# Autodesk Inventor assembly: Assembly_Cube_Lens_holder_v3
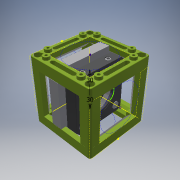
[picture p0: Inventor's stored thumbnail of the model, 180x180]
Saved by Autodesk Inventor 2019 (Build 230136000, 136)
## iProperties
Created: 2020-11-11
Part Number: Assembly_Cube_Lens_holder_v3
Document SubType Name: Assembly
Designer: marsikovabarbora
Author: marsikovabarbora
## Documents named in this file (4)
- C:\Users\UC2\Dropbox\UC2\02_CAD\INVENTOR\uc2_v3\Assembly_Cube_Thorlabs_Cage_v3.iam
- C:\Users\UC2\Dropbox\UC2\02_CAD\INVENTOR\uc2_v3\Assembly_Cube_empty_IM_v3.iam
- C:\Users\UC2\Dropbox\UC2\02_CAD\INVENTOR\uc2_v3\00_Thorlabs_Cage_CP33_M.ipt
- C:\Users\UC2\Dropbox\UC2\02_CAD\INVENTOR\uc2_v3\Imported Components\20_Insert_Thorlabs_holder_v3\20_Insert_Thorlabs_holder_v3.ipt
## Components (3 placed, 3 different names)
1. Assembly_Cube_empty_IM_v3:1 [sub-assembly] — Mate:1, Mate:2, Mate:3, Passend:5, Passend:6, Winkel:2
2. 00_Thorlabs_Cage_CP33_M:1 — Passend:4, Winkel:1, Fluchtend:1
3. 20_Insert_Thorlabs_holder_v3:1 — Passend:4, Winkel:1, Fluchtend:1, Passend:5, Passend:6, Winkel:2
## Relationships (9: Mate 6, Angle 2, Flush 1)
- Mate:1: Assembly_Cube_empty_IM_v3:1
- Mate:2: Assembly_Cube_empty_IM_v3:1
- Mate:3: Assembly_Cube_empty_IM_v3:1
- Passend:4 [Mate]: 00_Thorlabs_Cage_CP33_M:1 ↔ 20_Insert_Thorlabs_holder_v3:1
- Winkel:1 [Angle] (0 deg): 00_Thorlabs_Cage_CP33_M:1 ↔ 20_Insert_Thorlabs_holder_v3:1
- Fluchtend:1 [Flush]: 00_Thorlabs_Cage_CP33_M:1 ↔ 20_Insert_Thorlabs_holder_v3:1
- Passend:5 [Mate]: Assembly_Cube_empty_IM_v3:1 ↔ 20_Insert_Thorlabs_holder_v3:1
- Passend:6 [Mate]: Assembly_Cube_empty_IM_v3:1 ↔ 20_Insert_Thorlabs_holder_v3:1
- Winkel:2 [Angle] (0 deg): Assembly_Cube_empty_IM_v3:1 ↔ 20_Insert_Thorlabs_holder_v3:1
